# Autodesk Inventor assembly: v3.0
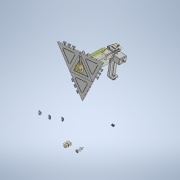
[picture p0: Inventor's stored thumbnail of the model, 180x180]
Saved by Autodesk Inventor 2022.3 (Build 263350000, 350)
## iProperties
Created: 2023-05-20
Part Number: v3.0
Document SubType Name: Assembly
Designer: Manuel Hueso Béjar
Author: Manuel Hueso Béjar
## Documents named in this file (19)
- C:\Users\Manuel Hueso Béjar\Desktop\3\2º Cuatrimestre\Robótica\2_Trabajo\CAD\v3.0\v3.0.iam
- C:\Users\Manuel Hueso Béjar\Desktop\3\2º Cuatrimestre\Robótica\2_Trabajo\CAD\v3.0\Base.ipt
- C:\Users\Manuel Hueso Béjar\Desktop\3\2º Cuatrimestre\Robótica\2_Trabajo\CAD\v3.0\Base2.ipt
- C:\Users\Manuel Hueso Béjar\Desktop\3\2º Cuatrimestre\Robótica\2_Trabajo\CAD\v3.0\DoveTail_Joint_1.ipt
- C:\Users\Manuel Hueso Béjar\Desktop\3\2º Cuatrimestre\Robótica\2_Trabajo\CAD\v3.0\Joint_Bearings.ipt
- C:\Users\Manuel Hueso Béjar\Desktop\3\2º Cuatrimestre\Robótica\2_Trabajo\CAD\v3.0\Joint_Tubes_1_1.ipt
- C:\Users\Manuel Hueso Béjar\Desktop\3\2º Cuatrimestre\Robótica\2_Trabajo\CAD\v3.0\Joint_Tubes_1_2.ipt
- C:\Users\Manuel Hueso Béjar\Desktop\3\2º Cuatrimestre\Robótica\2_Trabajo\CAD\v3.0\Potenciómetro.ipt
- C:\Users\Manuel Hueso Béjar\Desktop\3\2º Cuatrimestre\Robótica\2_Trabajo\CAD\v3.0\Rod_1.ipt
- C:\Users\Manuel Hueso Béjar\Desktop\3\2º Cuatrimestre\Robótica\2_Trabajo\CAD\v3.0\Tube_1_1.ipt
- C:\Users\Manuel Hueso Béjar\Desktop\3\2º Cuatrimestre\Robótica\2_Trabajo\CAD\v3.0\Tube_1_2.ipt
- C:\Users\Manuel Hueso Béjar\Desktop\3\2º Cuatrimestre\Robótica\2_Trabajo\CAD\v3.0\Tube_2.ipt
- C:\Users\Manuel Hueso Béjar\Desktop\3\2º Cuatrimestre\Robótica\2_Trabajo\CAD\v3.0\Tube_3.ipt
- C:\Users\Manuel Hueso Béjar\Downloads\rolling-bearing-lmxxuu-1.snapshot.6\roulement lmxxuu (ap203).ipt
- C:\Users\Manuel Hueso Béjar\Downloads\timing-pulley-gt2-16-teeth-5mm-bore-2.snapshot.7\GT2-16T\GT2_16T.ipt
- C:\Users\Manuel Hueso Béjar\Downloads\nema-17-motor-a-pasos-17hs4401-1-7amp-4kg-cm-1.snapshot.4\Nema 17 Motor a Pasos 17HS4401.iam
- C:\Users\Manuel Hueso Béjar\Desktop\3\2º Cuatrimestre\Robótica\2_Trabajo\CAD\v3.0\Tensor.ipt
- C:\Users\Manuel Hueso Béjar\Desktop\3\2º Cuatrimestre\Robótica\2_Trabajo\CAD\v3.0\Stepper_Closing_1.ipt
- C:\Users\Manuel Hueso Béjar\Desktop\3\2º Cuatrimestre\Robótica\2_Trabajo\CAD\v3.0\Stepper_Closing_2.ipt
## Components (26 placed, 18 different names)
1. Base:1 — Rigid:1, Rigid:2, Rigid:3, Rigid:4
2. Base2:1 — Rigid:1
3. Base2:2 — Rigid:2
4. Base2:3 — Rigid:3
5. DoveTail_Joint_1:1
6. DoveTail_Joint_1:2
7. DoveTail_Joint_1:3
8. Joint_Bearings:1 — Rigid:8, Rigid:9, Rigid:11, Rigid:13
9. Joint_Tubes_1_1:1 — Rigid:7, Rotational:3, Rotational:4
10. Joint_Tubes_1_2:1 — Rigid:6, Rigid:12
11. Potenciómetro:1
12. Rod_1:1 — Rotational:3, Cylindrical:1
13. Rod_1:2 — Rotational:4, Cylindrical:2
14. Tube_1_1:1 — Rotational:1, Rigid:5
15. Tube_1_2:1 — Rigid:5, Rigid:6, Rigid:7, Rigid:10
16. Tube_2:1 — Rotational:5
17. Tube_3:1
18. roulement lmxxuu (ap203):1 — Rigid:9, Cylindrical:2
19. roulement lmxxuu (ap203):2 — Rigid:8, Cylindrical:1
20. GT2_16T:1
21. Nema 17 Motor a Pasos 17HS4401:1 [sub-assembly] — Rigid:4, Rotational:1
22. Nema 17 Motor a Pasos 17HS4401:2 [sub-assembly] — Rigid:10, Rotational:6
23. Nema 17 Motor a Pasos 17HS4401:3 [sub-assembly] — Rigid:11, Rotational:5
24. Tensor:1 — Rigid:12
25. Stepper_Closing_1:1 — Rotational:6
26. Stepper_Closing_2:1 — Rigid:13
## Relationships (20: WeldJoint 13, RevoluteJoint 5, CylindricalJoint 2)
- Rigid:1 [WeldJoint]: Base:1 ↔ Base2:1
- Rigid:2 [WeldJoint]: Base:1 ↔ Base2:2
- Rigid:3 [WeldJoint]: Base:1 ↔ Base2:3
- Rigid:4 [WeldJoint]: Base:1 ↔ Nema 17 Motor a Pasos 17HS4401:1
- Rotational:1 [RevoluteJoint] (-2.25 mm): Tube_1_1:1 ↔ Nema 17 Motor a Pasos 17HS4401:1
- Rigid:5 [WeldJoint]: Tube_1_1:1 ↔ Tube_1_2:1
- Rigid:6 [WeldJoint]: Joint_Tubes_1_2:1 ↔ Tube_1_2:1
- Rigid:7 [WeldJoint]: Joint_Tubes_1_1:1 ↔ Tube_1_2:1
- Rotational:3 [RevoluteJoint] (-3 mm): Joint_Tubes_1_1:1 ↔ Rod_1:1
- Rotational:4 [RevoluteJoint] (-3 mm): Joint_Tubes_1_1:1 ↔ Rod_1:2
- Rigid:8 [WeldJoint]: Joint_Bearings:1 ↔ roulement lmxxuu (ap203):2
- Rigid:9 [WeldJoint]: Joint_Bearings:1 ↔ roulement lmxxuu (ap203):1
- Cylindrical:1: Rod_1:1 ↔ roulement lmxxuu (ap203):2
- Cylindrical:2: Rod_1:2 ↔ roulement lmxxuu (ap203):1
- Rigid:10 [WeldJoint]: Tube_1_2:1 ↔ Nema 17 Motor a Pasos 17HS4401:2
- Rigid:11 [WeldJoint]: Joint_Bearings:1 ↔ Nema 17 Motor a Pasos 17HS4401:3
- Rigid:12 [WeldJoint]: Joint_Tubes_1_2:1 ↔ Tensor:1
- Rotational:5 [RevoluteJoint] (-7.5 mm): Tube_2:1 ↔ Nema 17 Motor a Pasos 17HS4401:3
- Rotational:6 [RevoluteJoint]: Nema 17 Motor a Pasos 17HS4401:2 ↔ Stepper_Closing_1:1
- Rigid:13 [WeldJoint]: Joint_Bearings:1 ↔ Stepper_Closing_2:1
